# Autodesk Inventor assembly: axis5_6  compact
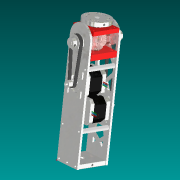
[picture p0: Inventor's stored thumbnail of the model, 180x180]
Saved by Autodesk Inventor 2020.3 (Build 243373000, 373)
## iProperties
Created: 2020-05-15
Part Number: axis5_6  compact
Document SubType Name: Assembly
Designer: stefa
Author: stefa
## Documents named in this file (12)
- C:\Users\Svend\OneDrive\Documents\GitHub\BeerMinder\3D-model\axis5_6\axis5_6  compact.iam
- C:\Users\Svend\OneDrive\Documents\GitHub\BeerMinder\3D-model\pulleys\GT2 Timing Pulley 36T - 8mm as.ipt
- C:\Users\Svend\OneDrive\Documents\GitHub\BeerMinder\3D-model\stepper motors\42BYG Stepper Motor.ipt
- C:\Users\Svend\OneDrive\Documents\GitHub\BeerMinder\3D-model\pulleys\GT2 Pulley 16T - 5mm as.ipt
- C:\Users\Svend\OneDrive\Documents\GitHub\BeerMinder\3D-model\axis5_6\bovenarm - links.ipt
- C:\Users\Svend\OneDrive\Documents\GitHub\BeerMinder\3D-model\bearings\lager 8mm - buiten 14 (sven 2 stuks).ipt
- C:\Users\Svend\OneDrive\Documents\GitHub\BeerMinder\3D-model\axis5_6\differential gearbox compact.iam
- C:\Users\Svend\OneDrive\Documents\GitHub\BeerMinder\3D-model\pulleys\tandriem32Tnaar16T_lengte280.ipt
- C:\Users\Svend\OneDrive\Documents\GitHub\BeerMinder\3D-model\pulleys\tandriem32Tnaar16T_lengte188.ipt
- C:\Users\Svend\OneDrive\Documents\GitHub\BeerMinder\3D-model\axis5_6\bovenarm - rechts.ipt
- C:\Users\Svend\OneDrive\Documents\GitHub\BeerMinder\3D-model\axis5_6\vul as platen.ipt
- C:\Users\Svend\OneDrive\Documents\GitHub\BeerMinder\3D-model\axis5_6\bevestegingsplaat axis5_6.ipt
## Components (18 placed, 11 different names)
1. tandriem32Tnaar16T_lengte280:1 — Mate:57, Mate:58, Mate:106, Mate:107
2. tandriem32Tnaar16T_lengte188:1 — Mate:60, Mate:89, Mate:94, Mate:100
3. 42BYG Stepper Motor:2 — Mate:96, Mate:108, Tangent:120, Tangent:121
4. bovenarm - links:1 — Angle:3, Flush:6, Mate:96, Mate:109, Mate:113, Flush:14, Mate:118, Tangent:120, Tangent:121, Mate:120, Mate:123, Mate:124, Mate:125, Mate:128
5. GT2 Timing Pulley 36T - 8mm as:6 — Mate:57, Mate:58, Mate:115
6. GT2 Timing Pulley 36T - 8mm as:7 — Mate:60, Mate:100, Mate:114
7. bovenarm - rechts:1 — Flush:6, Mate:99, Mate:102, Mate:112, Flush:13, Mate:117, Tangent:122, Tangent:123, Mate:121, Mate:122, Mate:126, Mate:127, Flush:15, Mate:129
8. GT2 Pulley 16T - 5mm as:2 — Mate:89, Mate:94, Mate:101, Mate:102
9. GT2 Pulley 16T - 5mm as:3 — Mate:106, Mate:107, Mate:108, Mate:109
10. 42BYG Stepper Motor:3 — Mate:99, Mate:101, Tangent:122, Tangent:123
11. lager 8mm - buiten 14 (sven 2 stuks):1 — Mate:112, Flush:13, Mate:119
12. lager 8mm - buiten 14 (sven 2 stuks):2 — Mate:113, Flush:14, Mate:116
13. differential gearbox compact:1 [sub-assembly] — Mate:114, Mate:115, Mate:116, Mate:117, Mate:118, Mate:119
14. vul as platen:1 — Mate:120, Mate:121
15. vul as platen:2 — Mate:124, Mate:126
16. vul as platen:3 — Mate:123, Mate:127
17. vul as platen:4 — Mate:122, Mate:125
18. bevestegingsplaat axis5_6:1 — Mate:128, Flush:15, Mate:129
## Relationships (41: Mate 32, Flush 4, Tangent 4, Angle 1)
- Angle:3 (0 deg): bovenarm - links:1
- Mate:57 (0.5 mm): tandriem32Tnaar16T_lengte280:1 ↔ GT2 Timing Pulley 36T - 8mm as:6
- Mate:58: tandriem32Tnaar16T_lengte280:1 ↔ GT2 Timing Pulley 36T - 8mm as:6
- Mate:60 (0.5 mm): tandriem32Tnaar16T_lengte188:1 ↔ GT2 Timing Pulley 36T - 8mm as:7
- Flush:6: bovenarm - links:1 ↔ bovenarm - rechts:1
- Mate:89 (0.5 mm): tandriem32Tnaar16T_lengte188:1 ↔ GT2 Pulley 16T - 5mm as:2
- Mate:94: tandriem32Tnaar16T_lengte188:1 ↔ GT2 Pulley 16T - 5mm as:2
- Mate:96: 42BYG Stepper Motor:2 ↔ bovenarm - links:1
- Mate:99: bovenarm - rechts:1 ↔ 42BYG Stepper Motor:3
- Mate:100: tandriem32Tnaar16T_lengte188:1 ↔ GT2 Timing Pulley 36T - 8mm as:7
- Mate:101: GT2 Pulley 16T - 5mm as:2 ↔ 42BYG Stepper Motor:3
- Mate:102 (2 mm): bovenarm - rechts:1 ↔ GT2 Pulley 16T - 5mm as:2
- Mate:106: tandriem32Tnaar16T_lengte280:1 ↔ GT2 Pulley 16T - 5mm as:3
- Mate:107 (0.5 mm): tandriem32Tnaar16T_lengte280:1 ↔ GT2 Pulley 16T - 5mm as:3
- Mate:108: 42BYG Stepper Motor:2 ↔ GT2 Pulley 16T - 5mm as:3
- Mate:109 (2 mm): bovenarm - links:1 ↔ GT2 Pulley 16T - 5mm as:3
- Mate:112: bovenarm - rechts:1 ↔ lager 8mm - buiten 14 (sven 2 stuks):1
- Flush:13: bovenarm - rechts:1 ↔ lager 8mm - buiten 14 (sven 2 stuks):1
- Mate:113: bovenarm - links:1 ↔ lager 8mm - buiten 14 (sven 2 stuks):2
- Flush:14: bovenarm - links:1 ↔ lager 8mm - buiten 14 (sven 2 stuks):2
- Mate:114: GT2 Timing Pulley 36T - 8mm as:7 ↔ differential gearbox compact:1
- Mate:115: GT2 Timing Pulley 36T - 8mm as:6 ↔ differential gearbox compact:1
- Mate:116: lager 8mm - buiten 14 (sven 2 stuks):2 ↔ differential gearbox compact:1
- Mate:117 (1 mm): bovenarm - rechts:1 ↔ differential gearbox compact:1
- Mate:118 (1 mm): bovenarm - links:1 ↔ differential gearbox compact:1
- Tangent:120 (0.3 mm): 42BYG Stepper Motor:2 ↔ bovenarm - links:1
- Tangent:121 (0.3 mm): 42BYG Stepper Motor:2 ↔ bovenarm - links:1
- Mate:119: lager 8mm - buiten 14 (sven 2 stuks):1 ↔ differential gearbox compact:1
- Tangent:122 (0.3 mm): bovenarm - rechts:1 ↔ 42BYG Stepper Motor:3
- Tangent:123 (0.3 mm): bovenarm - rechts:1 ↔ 42BYG Stepper Motor:3
- Mate:120: bovenarm - links:1 ↔ vul as platen:1
- Mate:121: bovenarm - rechts:1 ↔ vul as platen:1
- Mate:122: bovenarm - rechts:1 ↔ vul as platen:4
- Mate:123: bovenarm - links:1 ↔ vul as platen:3
- Mate:124: bovenarm - links:1 ↔ vul as platen:2
- Mate:125: bovenarm - links:1 ↔ vul as platen:4
- Mate:126: bovenarm - rechts:1 ↔ vul as platen:2
- Mate:127: bovenarm - rechts:1 ↔ vul as platen:3
- Mate:128: bovenarm - links:1 ↔ bevestegingsplaat axis5_6:1
- Flush:15: bovenarm - rechts:1 ↔ bevestegingsplaat axis5_6:1
- Mate:129: bovenarm - rechts:1 ↔ bevestegingsplaat axis5_6:1
